# Autodesk Inventor assembly: !structure_mirrored
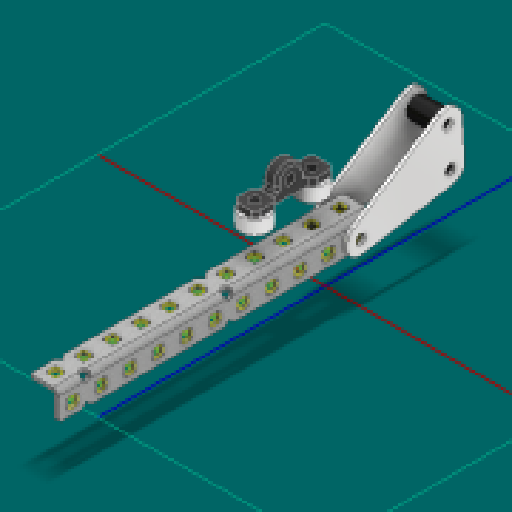
[picture p0: Inventor's stored thumbnail of the model, 512x512]
Saved by Autodesk Inventor 2025 (Build 290162000, 162)
## iProperties
Created: 2024-08-19
Part Number: !structure_mirrored
Document SubType Name: Assembly
Designer: averey
Author: averey
## Documents named in this file (10)
- C:\Users\avere\vex_robotics_high_stakes\hardware\cad\ATLAS\intake\second_stage\structure_mirrored\!structure_mirrored.iam
- C:\Users\avere\vex_robotics_high_stakes\hardware\cad\ATLAS\intake\second_stage\structure_mirrored\gusset_mirrored.ipt
- C:\Users\avere\vex_robotics_high_stakes\hardware\cad\ATLAS\intake\second_stage\structure_mirrored\Alu Angle 1x1x11_mirrored.ipt
- C:\Users\avere\vex_robotics_high_stakes\hardware\cad\VEX-CAD-Inventor\Motion\Spacers\Spacer Nylon .375 OD\NSpacer .375 OD x .500.ipt
- C:\Users\avere\vex_robotics_high_stakes\hardware\cad\VEX-CAD-Inventor\Motion\Spacers\Spacer Nylon .375 OD.ipt
- C:\Users\avere\vex_robotics_high_stakes\hardware\cad\VEX-CAD-Inventor\Motion\Spacers\Washer Steel\SWasher .375 OD x .062500.ipt
- C:\Users\avere\vex_robotics_high_stakes\hardware\cad\VEX-CAD-Inventor\Motion\Spacers\Washer Steel.ipt
- C:\Users\avere\vex_robotics_high_stakes\hardware\cad\VEX-CAD-Inventor\Motion\Shaft LS\LS Pillow Bearing Block.ipt
- C:\Users\avere\vex_robotics_high_stakes\hardware\cad\VEX-CAD-Inventor\Motion\Spacers\Spacer Nylon .500 OD\NSpacer White .500 OD x .250.ipt
- C:\Users\avere\vex_robotics_high_stakes\hardware\cad\VEX-CAD-Inventor\Motion\Spacers\Spacer Nylon .500 OD.ipt
## Components (10 placed, 6 different names)
1. gusset_mirrored:1 — Insert:1, Mate:1, Insert:4, Insert:6, Insert:11, Insert:15
2. gusset_mirrored:2 — Mate:2, Insert:1, Mate:1, Angle:1
3. Alu Angle 1x1x11_mirrored:1 — Angle:1, Angle:2, Insert:15, Insert:16, Mate:3
4. NSpacer .375 OD x .500:1 — Insert:4
5. NSpacer .375 OD x .500:2 — Insert:6
6. NSpacer .375 OD x .500:3 — Insert:10
7. SWasher .375 OD x .062500:2 — Insert:10, Insert:11
8. LS Pillow Bearing Block:1 — Insert:12, Insert:14
9. NSpacer White .500 OD x .250:1 — Insert:14, Mate:3
10. NSpacer White .500 OD x .250:2 — Insert:12, Insert:16
## Relationships (14: Insert 9, Mate 3, Angle 2)
- Mate:2: gusset_mirrored:2
- Insert:1 (14.2875 mm): gusset_mirrored:1 ↔ gusset_mirrored:2
- Mate:1: gusset_mirrored:1 ↔ gusset_mirrored:2
- Angle:1 (-9.6283 deg): gusset_mirrored:2 ↔ Alu Angle 1x1x11_mirrored:1
- Angle:2 (0 deg): Alu Angle 1x1x11_mirrored:1
- Insert:4: gusset_mirrored:1 ↔ NSpacer .375 OD x .500:1
- Insert:6: gusset_mirrored:1 ↔ NSpacer .375 OD x .500:2
- Insert:10: NSpacer .375 OD x .500:3 ↔ SWasher .375 OD x .062500:2
- Insert:11: gusset_mirrored:1 ↔ SWasher .375 OD x .062500:2
- Insert:12: LS Pillow Bearing Block:1 ↔ NSpacer White .500 OD x .250:2
- Insert:14: LS Pillow Bearing Block:1 ↔ NSpacer White .500 OD x .250:1
- Insert:15: gusset_mirrored:1 ↔ Alu Angle 1x1x11_mirrored:1
- Insert:16 (12.7 mm): Alu Angle 1x1x11_mirrored:1 ↔ NSpacer White .500 OD x .250:2
- Mate:3: Alu Angle 1x1x11_mirrored:1 ↔ NSpacer White .500 OD x .250:1
